# Autodesk Inventor assembly: 組合4
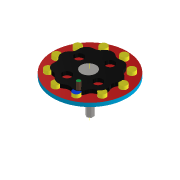
[picture p0: Inventor's stored thumbnail of the model, 180x180]
Saved by Autodesk Inventor 2022 (Build 260153000, 153)
## iProperties
Created: 2023-10-31
Part Number: 組合4
Document SubType Name: Assembly
Designer: JOU
Author: JOU
## Documents named in this file (4)
- C:\Users\JOU\Desktop\git\Special-project\Cycloidal Gear\組合4.iam
- C:\Users\JOU\Desktop\git\Special-project\Cycloidal Gear\180219-Disk.ipt
- C:\Users\JOU\Desktop\git\Special-project\Cycloidal Gear\180219-InputShaft.ipt
- C:\Users\JOU\Desktop\git\Special-project\Cycloidal Gear\180219-Base.ipt
## Components (3 placed, 3 different names)
1. 180219-Disk:1
2. 180219-InputShaft:1
3. 180219-Base:1 — 角度:1
## Relationships (5: Mate 3, Flush 1, Angle 1)
- [Mate]: 180219-InputShaft:1 ↔ 180219-Base:1
- [Mate]: 180219-Disk:1 ↔ 180219-InputShaft:1
- [Flush]: 180219-Disk:1 ↔ 180219-InputShaft:1
- [Mate]: 180219-Disk:1 ↔ 180219-Base:1
- 角度:1 [Angle] (1347 deg): 180219-Base:1
## Named parameters: d1_d2 = 0 mm, d2_d3 = 0 mm
